# Autodesk Inventor assembly: UpperBumperUnit
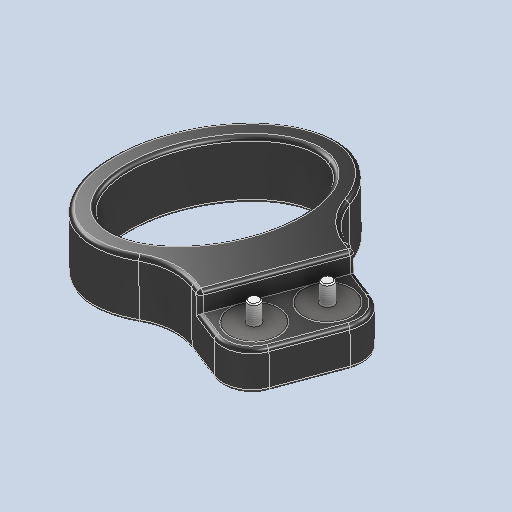
[picture p0: Inventor's stored thumbnail of the model, 512x512]
Saved by Autodesk Inventor 2024.2 (Build 282272000, 272)
## iProperties
Created: 2024-04-14
Part Number: UpperBumperUnit
Document SubType Name: Assembly
Designer: Masato Kubotera
Author: Masato Kubotera
## Documents named in this file (5)
- C:\Users\masato\OneDrive - Chiba Institute of Technology\CIT Brains\RoboCup2024\Mechanic\SUSTAINA-OP2-DEV - 作業\NativeFiles\Boby\Torso\TorsoBumpers\UpperBumperUnit.iam
- C:\Users\masato\OneDrive - Chiba Institute of Technology\CIT Brains\RoboCup2024\Mechanic\SUSTAINA-OP2-DEV - 作業\NativeFiles\Boby\COTS\Washers\Metal\UUW-0312-10H.ipt
- C:\Users\masato\OneDrive - Chiba Institute of Technology\CIT Brains\RoboCup2024\Mechanic\SUSTAINA-OP2-DEV - 作業\NativeFiles\Boby\Torso\TorsoBumpers\TorsoFrontBumper.ipt
- C:\Users\masato\OneDrive - Chiba Institute of Technology\CIT Brains\RoboCup2024\Mechanic\SUSTAINA-OP2-DEV - 作業\NativeFiles\Boby\COTS\Spacers\BRU-309S.ipt
- C:\Users\masato\OneDrive - Chiba Institute of Technology\CIT Brains\RoboCup2024\Mechanic\SUSTAINA-OP2-DEV - 作業\NativeFiles\Boby\COTS\Screws\LowHeadCapScrew\ULC-0306.ipt
## Components (9 placed, 4 different names)
1. UUW-0312-10H:1 — Insert:3, Insert:5
2. UUW-0312-10H:2 — Insert:4, Insert:6
3. TorsoFrontBumper:1 — Insert:3, Insert:4, Insert:7, Insert:8
4. UUW-0312-10H:3 — Insert:1, Insert:7
5. BRU-309S:2 — Insert:5
6. BRU-309S:1 — Insert:6
7. UUW-0312-10H:4 — Insert:2, Insert:8
8. ULC-0306:1 — Insert:1
9. ULC-0306:2 — Insert:2
## Relationships (8: Insert 8)
- Insert:1: UUW-0312-10H:3 ↔ ULC-0306:1
- Insert:2: UUW-0312-10H:4 ↔ ULC-0306:2
- Insert:3: UUW-0312-10H:1 ↔ TorsoFrontBumper:1
- Insert:4: UUW-0312-10H:2 ↔ TorsoFrontBumper:1
- Insert:5: UUW-0312-10H:1 ↔ BRU-309S:2
- Insert:6: UUW-0312-10H:2 ↔ BRU-309S:1
- Insert:7: TorsoFrontBumper:1 ↔ UUW-0312-10H:3
- Insert:8: TorsoFrontBumper:1 ↔ UUW-0312-10H:4
